# Autodesk Inventor assembly: SensorAssembly
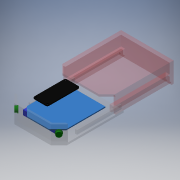
[picture p0: Inventor's stored thumbnail of the model, 180x180]
Saved by Autodesk Inventor 2018 (Build 220112000, 112)
## iProperties
Created: 2019-10-14
Part Number: SensorAssembly
Document SubType Name: Assembly
Designer: jklei
Author: jklei
## Documents named in this file (7)
- C:\Users\jklei\Desktop\Wildfire-Detector\CAD\SensorAssembly.iam
- C:\Users\jklei\Desktop\Wildfire-Detector\CAD\2829 Adafruit Feather Bluefruit 32u4.ipt
- C:\Users\jklei\Desktop\Wildfire-Detector\CAD\sensor.ipt
- C:\Users\jklei\Desktop\Wildfire-Detector\CAD\bottom-housing.ipt
- C:\Users\jklei\Desktop\Wildfire-Detector\CAD\top-slider.ipt
- C:\Users\jklei\Desktop\Wildfire-Detector\CAD\PCB.ipt
- C:\Users\jklei\Desktop\Wildfire-Detector\CAD\Battery.ipt
## Components (7 placed, 6 different names)
1. 2829 Adafruit Feather Bluefruit 32u4:1 — Flush:3, Mate:15, Flush:4
2. sensor:1 — Insert:2
3. sensor:2 — Insert:1
4. bottom-housing:1 — Flush:1, Mate:6, Insert:1, Insert:2, Mate:9, Mate:10, Mate:11, Mate:13, Mate:14
5. top-slider:1 — Flush:1, Mate:6
6. PCB:1 — Flush:3, Mate:9, Mate:10, Mate:12, Mate:15, Flush:4
7. Battery:1 — Mate:11, Mate:12, Mate:13, Mate:14
## Relationships (13: Mate 8, Flush 3, Insert 2)
- Flush:1: bottom-housing:1 ↔ top-slider:1
- Mate:6: bottom-housing:1 ↔ top-slider:1
- Insert:1: sensor:2 ↔ bottom-housing:1
- Insert:2: sensor:1 ↔ bottom-housing:1
- Flush:3 (3.175 mm): 2829 Adafruit Feather Bluefruit 32u4:1 ↔ PCB:1
- Mate:9 (3.81 mm): bottom-housing:1 ↔ PCB:1
- Mate:10 (5.08 mm): bottom-housing:1 ↔ PCB:1
- Mate:11: bottom-housing:1 ↔ Battery:1
- Mate:12: PCB:1 ↔ Battery:1
- Mate:13 (3.81 mm): bottom-housing:1 ↔ Battery:1
- Mate:14 (12.7 mm): bottom-housing:1 ↔ Battery:1
- Mate:15 (8.382 mm): 2829 Adafruit Feather Bluefruit 32u4:1 ↔ PCB:1
- Flush:4 (2.54 mm): 2829 Adafruit Feather Bluefruit 32u4:1 ↔ PCB:1
